# Autodesk Inventor assembly: ARM_058_BottomRoller
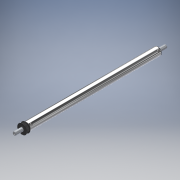
[picture p0: Inventor's stored thumbnail of the model, 180x180]
Saved by Autodesk Inventor 2018.3 (Build 223284000, 284)
## iProperties
Created: 2020-02-08
Part Number: ARM_058_BottomRoller
Document SubType Name: Assembly
Designer: 22turnmaxw
Mass: 304.474 g
Surface Area: 1325.64 cm^2
Volume: 125.504 cm^3
Density: 2.42601 g/cm^3
Author: 22turnmaxw
## Documents named in this file (8)
- C:\Users\22barlalex\Documents\GrabCAD\Infinite Recharge 2020\Build season\ARM_058_BottomRoller.iam
- C:\Users\22barlalex\Documents\GrabCAD\Infinite Recharge 2020\Build season\ARM_015_VersaRoller_Hub_1_2_Hex_Bore_x_1-1_8_OD_Aluminum_217-5895.ipt
- C:\Users\22barlalex\Documents\GrabCAD\Infinite Recharge 2020\Build season\ARM_034_36Tx9mm3mmPitchPulley.ipt
- C:\Users\22barlalex\Documents\GrabCAD\Infinite Recharge 2020\Build season\ARM_027_ANSI B18.3 - 5_16-18 UNC - UNC - 0.5.ipt
- C:\Users\22barlalex\Documents\GrabCAD\Infinite Recharge 2020\Build season\ARM_028_ANSI B18.3 - 10-24 UNC - UNC - 0.1875.ipt
- C:\Users\22barlalex\Documents\GrabCAD\Infinite Recharge 2020\Build season\ARM_059_BottomRollerHexInserts.ipt
- C:\Users\22barlalex\Documents\GrabCAD\Infinite Recharge 2020\Build season\ARM_065_BottomRollerHexInsertsRight.ipt
- C:\Users\22barlalex\Documents\GrabCAD\Infinite Recharge 2020\Build season\ARM_081_BottomRollerTube.ipt
## Components (12 placed, 7 different names)
1. ARM_015_VersaRoller_Hub_1_2_Hex_Bore_x_1-1_8_OD_Aluminum_217-5895:1 — Mate:46, Mate:47
2. ARM_015_VersaRoller_Hub_1_2_Hex_Bore_x_1-1_8_OD_Aluminum_217-5895:2 — Mate:51, Mate:54, Mate:55, Mate:57
3. ARM_034_36Tx9mm3mmPitchPulley:1 — Mate:47, Mate:48, Mate:53
4. Hexagon Socket Button Head Cap Screw - Inch 5/16 - 18 x 1/2:2 — Mate:44, Mate:45
5. Hexagon Socket Button Head Cap Screw - Inch 10 - 24 x 3/16:1 — Mate:54, Tangent:1, Mate:56
6. Hexagon Socket Button Head Cap Screw - Inch 10 - 24 x 3/16:2 — Mate:59, Tangent:2
7. Hexagon Socket Button Head Cap Screw - Inch 10 - 24 x 3/16:3 — Mate:52
8. Hexagon Socket Button Head Cap Screw - Inch 10 - 24 x 3/16:4
9. Hexagon Socket Button Head Cap Screw - Inch 5/16 - 18 x 1/2:3 — Mate:49, Mate:50
10. ARM_059_BottomRollerHexInserts:2 — Mate:44, Mate:45, Mate:46, Mate:48
11. ARM_065_BottomRollerHexInsertsRight:1 — Mate:49, Mate:50, Mate:51, Mate:57, Mate:58
12. ARM_081_BottomRollerTube:1 — Mate:52, Mate:53, Mate:55, Tangent:1, Mate:56, Mate:58, Mate:59, Tangent:2
## Relationships (18: Mate 16, Tangent 2)
- Mate:44: Hexagon Socket Button Head Cap Screw - Inch 5/16 - 18 x 1/2:2 ↔ ARM_059_BottomRollerHexInserts:2
- Mate:45: Hexagon Socket Button Head Cap Screw - Inch 5/16 - 18 x 1/2:2 ↔ ARM_059_BottomRollerHexInserts:2
- Mate:46: ARM_015_VersaRoller_Hub_1_2_Hex_Bore_x_1-1_8_OD_Aluminum_217-5895:1 ↔ ARM_059_BottomRollerHexInserts:2
- Mate:47: ARM_015_VersaRoller_Hub_1_2_Hex_Bore_x_1-1_8_OD_Aluminum_217-5895:1 ↔ ARM_034_36Tx9mm3mmPitchPulley:1
- Mate:48: ARM_034_36Tx9mm3mmPitchPulley:1 ↔ ARM_059_BottomRollerHexInserts:2
- Mate:49: Hexagon Socket Button Head Cap Screw - Inch 5/16 - 18 x 1/2:3 ↔ ARM_065_BottomRollerHexInsertsRight:1
- Mate:50: Hexagon Socket Button Head Cap Screw - Inch 5/16 - 18 x 1/2:3 ↔ ARM_065_BottomRollerHexInsertsRight:1
- Mate:51: ARM_015_VersaRoller_Hub_1_2_Hex_Bore_x_1-1_8_OD_Aluminum_217-5895:2 ↔ ARM_065_BottomRollerHexInsertsRight:1
- Mate:52: Hexagon Socket Button Head Cap Screw - Inch 10 - 24 x 3/16:3 ↔ ARM_081_BottomRollerTube:1
- Mate:53: ARM_034_36Tx9mm3mmPitchPulley:1 ↔ ARM_081_BottomRollerTube:1
- Mate:54: ARM_015_VersaRoller_Hub_1_2_Hex_Bore_x_1-1_8_OD_Aluminum_217-5895:2 ↔ Hexagon Socket Button Head Cap Screw - Inch 10 - 24 x 3/16:1
- Mate:55: ARM_015_VersaRoller_Hub_1_2_Hex_Bore_x_1-1_8_OD_Aluminum_217-5895:2 ↔ ARM_081_BottomRollerTube:1
- Tangent:1: Hexagon Socket Button Head Cap Screw - Inch 10 - 24 x 3/16:1 ↔ ARM_081_BottomRollerTube:1
- Mate:56: Hexagon Socket Button Head Cap Screw - Inch 10 - 24 x 3/16:1 ↔ ARM_081_BottomRollerTube:1
- Mate:57: ARM_015_VersaRoller_Hub_1_2_Hex_Bore_x_1-1_8_OD_Aluminum_217-5895:2 ↔ ARM_065_BottomRollerHexInsertsRight:1
- Mate:58: ARM_065_BottomRollerHexInsertsRight:1 ↔ ARM_081_BottomRollerTube:1
- Mate:59: Hexagon Socket Button Head Cap Screw - Inch 10 - 24 x 3/16:2 ↔ ARM_081_BottomRollerTube:1
- Tangent:2: Hexagon Socket Button Head Cap Screw - Inch 10 - 24 x 3/16:2 ↔ ARM_081_BottomRollerTube:1
